# Autodesk Inventor assembly: компановка емкость
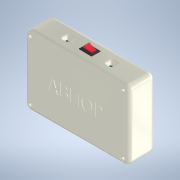
[picture p0: Inventor's stored thumbnail of the model, 180x180]
Saved by Autodesk Inventor 2021 (Build 250183000, 183)
## iProperties
Created: 2023-02-13
Part Number: компановка емкость
Document SubType Name: Assembly
Designer: Tasya
Author: Tasya
## Documents named in this file (8)
- C:\Users\Tasya\Desktop\теплица\3D модели\Сборки iam\емкость\компановка емкость.iam
- C:\Users\Tasya\Desktop\теплица\grabcad\Wemos_D1_mini.ipt
- C:\Users\Tasya\Desktop\теплица\grabcad\реле.ipt
- C:\Users\Tasya\Desktop\теплица\grabcad\конденсатор.ipt
- C:\Users\Tasya\Desktop\теплица\grabcad\Switch on off.ipt
- C:\Users\Tasya\Desktop\теплица\емкость\корпус емкость.ipt
- C:\Users\Tasya\Desktop\теплица\емкость\столбики.ipt
- C:\Users\Tasya\Desktop\теплица\кронштейн wemos.ipt
## Components (8 placed, 7 different names)
1. Wemos_D1_mini:1 — Совмещение:12, Заподлицо:14, Заподлицо:15
2. реле:1 — Совмещение:5, Совмещение:6, Совмещение:7, Совмещение:8, Совмещение:9, Совмещение:10
3. конденсатор:1
4. Switch on off:1 — Совмещение:4
5. корпус емкость:1 — Совмещение:4, Совмещение:5, Совмещение:6, Совмещение:7, Совмещение:11
6. столбики:1 — Совмещение:8, Совмещение:10, Совмещение:13, Совмещение:14
7. столбики:2 — Совмещение:9, Совмещение:11, Совмещение:15
8. кронштейн wemos:1 — Совмещение:12, Заподлицо:14, Заподлицо:15, Совмещение:13, Совмещение:14, Совмещение:15
## Relationships (14: Mate 12, Flush 2)
- Совмещение:4 [Mate]: Switch on off:1 ↔ корпус емкость:1
- Совмещение:5 [Mate]: реле:1 ↔ корпус емкость:1
- Совмещение:6 [Mate]: реле:1 ↔ корпус емкость:1
- Совмещение:7 [Mate]: реле:1 ↔ корпус емкость:1
- Совмещение:8 [Mate]: реле:1 ↔ столбики:1
- Совмещение:9 [Mate]: реле:1 ↔ столбики:2
- Совмещение:10 [Mate]: реле:1 ↔ столбики:1
- Совмещение:11 [Mate]: корпус емкость:1 ↔ столбики:2
- Совмещение:12 [Mate]: Wemos_D1_mini:1 ↔ кронштейн wemos:1
- Заподлицо:14 [Flush]: Wemos_D1_mini:1 ↔ кронштейн wemos:1
- Заподлицо:15 [Flush] (25 mm): Wemos_D1_mini:1 ↔ кронштейн wemos:1
- Совмещение:13 [Mate]: столбики:1 ↔ кронштейн wemos:1
- Совмещение:14 [Mate]: столбики:1 ↔ кронштейн wemos:1
- Совмещение:15 [Mate]: столбики:2 ↔ кронштейн wemos:1
